# Autodesk Inventor assembly: PlateWithHinges
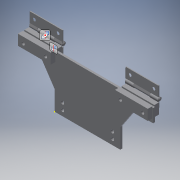
[picture p0: Inventor's stored thumbnail of the model, 180x180]
Saved by Autodesk Inventor 2017 (Build 210142000, 142)
## iProperties
Created: 2017-04-06
Part Number: PlateWithHinges
Document SubType Name: Assembly
Designer: s4461999
Author: s4461999
## Documents named in this file (4)
- U:\CAD\PlateWithHinges.iam
- U:\CAD\plate.ipt
- U:\CAD\adjustmentHingePlate.ipt
- U:\CAD\Hinge\SierraPacific-BH7015ZN.ipt
## Components (7 placed, 3 different names)
1. plate:1 — Mate:1, Mate:2, Mate:3, Mate:4
2. adjustmentHingePlate:1 — Mate:2, Mate:8, Mate:10
3. adjustmentHingePlate:2 — Mate:1, Mate:5, Mate:6, Mate:7
4. adjustmentHingePlate:3 — Mate:4
5. adjustmentHingePlate:4 — Mate:3
6. SierraPacific-BH7015ZN:1 — Mate:5, Mate:6, Mate:7, Mate:9
7. SierraPacific-BH7015ZN:3 — Mate:8, Mate:9, Mate:10
## Relationships (10: Mate 10)
- Mate:1: plate:1 ↔ adjustmentHingePlate:2
- Mate:2: plate:1 ↔ adjustmentHingePlate:1
- Mate:3: plate:1 ↔ adjustmentHingePlate:4
- Mate:4: plate:1 ↔ adjustmentHingePlate:3
- Mate:5: adjustmentHingePlate:2 ↔ SierraPacific-BH7015ZN:1
- Mate:6: adjustmentHingePlate:2 ↔ SierraPacific-BH7015ZN:1
- Mate:7 (2.07 mm): adjustmentHingePlate:2 ↔ SierraPacific-BH7015ZN:1
- Mate:8: adjustmentHingePlate:1 ↔ SierraPacific-BH7015ZN:3
- Mate:9: SierraPacific-BH7015ZN:1 ↔ SierraPacific-BH7015ZN:3
- Mate:10: adjustmentHingePlate:1 ↔ SierraPacific-BH7015ZN:3
